# Autodesk Inventor assembly: Cube
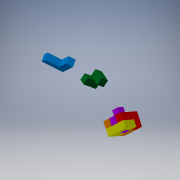
[picture p0: Inventor's stored thumbnail of the model, 180x180]
Saved by Autodesk Inventor 2017 (Build 210142000, 142)
## iProperties
Created: 2016-11-02
Part Number: Cube
Document SubType Name: Assembly
Designer: rbibb
Author: rbibb
## Documents named in this file (7)
- A:\rbibb\Desktop\Cube.iam
- A:\rbibb\Desktop\Blue part.ipt
- A:\rbibb\Desktop\Green part.ipt
- A:\rbibb\Desktop\Orange part.ipt
- A:\rbibb\Desktop\Purple part.ipt
- A:\rbibb\Desktop\Red part.ipt
- A:\rbibb\Desktop\Yellow part.ipt
## Components (6 placed, 6 different names)
1. Blue part:1
2. Green part:1
3. Orange part:1 — Mate:5, Mate:6, Flush:3
4. Purple part:1 — Mate:3, Mate:4, Flush:2, Mate:5, Flush:3
5. Red part:1 — Mate:1, Mate:2, Flush:1, Mate:6
6. Yellow part:1 — Mate:1, Mate:2, Flush:1, Mate:3, Mate:4, Flush:2
## Relationships (9: Mate 6, Flush 3)
- Mate:1: Red part:1 ↔ Yellow part:1
- Mate:2: Red part:1 ↔ Yellow part:1
- Flush:1: Red part:1 ↔ Yellow part:1
- Mate:3: Purple part:1 ↔ Yellow part:1
- Mate:4: Purple part:1 ↔ Yellow part:1
- Flush:2: Purple part:1 ↔ Yellow part:1
- Mate:5: Orange part:1 ↔ Purple part:1
- Mate:6: Orange part:1 ↔ Red part:1
- Flush:3: Orange part:1 ↔ Purple part:1
